# Autodesk Inventor assembly: 3.25 Omni AS, No Insert_MIR
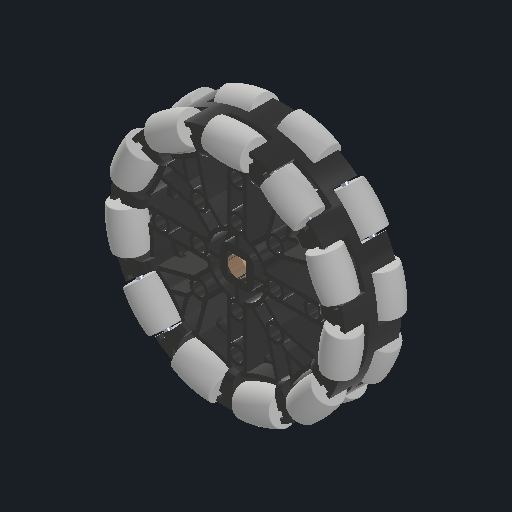
[picture p0: Inventor's stored thumbnail of the model, 512x512]
Saved by Autodesk Inventor 2026.1 (Build 301233000, 233)
## iProperties
Created: 2022-08-02
Part Number: 3.25 Omni AS, No Insert_MIR
Document SubType Name: Assembly
Designer: roejo
Author: ylu12
## Documents named in this file (2)
- C:\Users\roejo\OneDrive\Documents\7700RKalahariCAD\Library\VEX-CAD-Inventor-1.4.2\Motion\Wheels\Omni Wheel\3.25 Omni AS, No Insert_MIR.iam
- C:\Users\roejo\OneDrive\Documents\7700RKalahariCAD\Library\VEX-CAD-Inventor-1.4.2\Motion\Wheels\Reference Files\3.25 Omni Antistatic_MIR.ipt
## Components (1 placed, 1 different names)
1. 3.25 Omni Antistatic_MIR:1 — Mate:12, Mate:11, Flush:6
## Relationships (3: Mate 2, Flush 1)
- Mate:12: 3.25 Omni Antistatic_MIR:1
- Mate:11: 3.25 Omni Antistatic_MIR:1
- Flush:6: 3.25 Omni Antistatic_MIR:1
